# Autodesk Inventor assembly: Stadio3
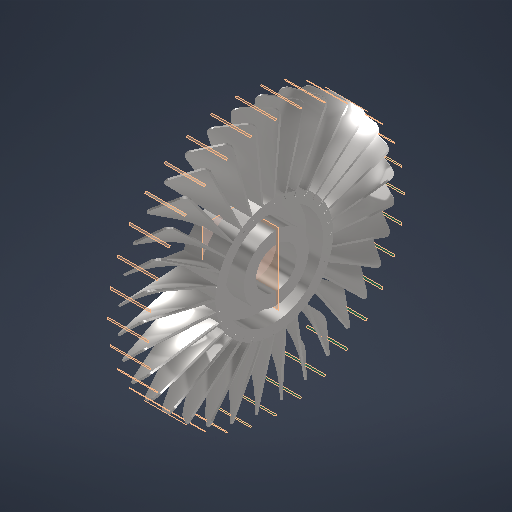
[picture p0: Inventor's stored thumbnail of the model, 512x512]
Saved by Autodesk Inventor 2026.2 (Build 302298010, 298A)
## iProperties
Created: 2026-04-23
Part Number: Stadio3
Document SubType Name: Assembly
Designer: Yan
Author: Yan
## Documents named in this file (3)
- C:\Users\Yan\Desktop\Turbina\Stadio3.iam
- C:\Users\Yan\Desktop\Turbina\DiscoPaleSatdio3-DimensioniAprossimate.ipt
- C:\Users\Yan\Desktop\Turbina\PalaStadio3.ipt
## Components (33 placed, 2 different names)
1. DiscoPaleSatdio3-DimensioniAprossimate:1 — Mate:1, Mate:3, Mate:4, Mate:5, Mate:6, Mate:7, Mate:8, Mate:9, Mate:10, Mate:11, Mate:12, Mate:13, Mate:14, Mate:15, Mate:16, Mate:17, Mate:18, Mate:19, Mate:20, Mate:21, Mate:22, Mate:23, Mate:24, Mate:25, Mate:26, Mate:27, Mate:28, Mate:29, Mate:30, Mate:31, Mate:32, Mate:33, Mate:34, Mate:35, Mate:36, Mate:37, Mate:40, Mate:41, Mate:42, Mate:43, Mate:44, Mate:45, Mate:46, Mate:47, Mate:48, Mate:49, Mate:50, Mate:51, Mate:52, Mate:53, Mate:54, Mate:55, Mate:56, Mate:57, Mate:58, Mate:59, Mate:60, Mate:61, Mate:62, Mate:63, Mate:64, Mate:65, Mate:66, Flush:1
2. PalaStadio3:1 — Mate:1, Mate:16, Flush:21
3. PalaStadio3:2 — Mate:30, Mate:31, Flush:20
4. PalaStadio3:3 — Mate:3, Mate:17, Flush:19
5. PalaStadio3:4 — Mate:4, Mate:18, Flush:18
6. PalaStadio3:5 — Mate:5, Mate:19, Flush:17
7. PalaStadio3:6 — Mate:6, Mate:20, Flush:16
8. PalaStadio3:7 — Mate:7, Mate:21, Flush:15
9. PalaStadio3:8 — Mate:8, Mate:22, Flush:14
10. PalaStadio3:9 — Mate:9, Mate:23, Flush:13
11. PalaStadio3:10 — Mate:10, Mate:24, Flush:12
12. PalaStadio3:11 — Mate:11, Mate:25, Flush:11
13. PalaStadio3:12 — Mate:58, Mate:59, Flush:32
14. PalaStadio3:13 — Mate:60, Mate:66, Flush:1, Flush:2, Flush:3, Flush:4, Flush:5, Flush:6, Flush:7, Flush:8, Flush:9, Flush:10, Flush:11, Flush:12, Flush:13, Flush:14, Flush:15, Flush:16, Flush:17, Flush:18, Flush:19, Flush:20, Flush:21, Flush:22, Flush:23, Flush:24, Flush:25, Flush:26, Flush:27, Flush:28, Flush:29, Flush:30, Flush:31, Flush:32
15. PalaStadio3:14 — Mate:37, Mate:61, Flush:2
16. PalaStadio3:15 — Mate:35, Mate:63, Flush:4
17. PalaStadio3:16 — Mate:36, Mate:64, Flush:3
18. PalaStadio3:17 — Mate:34, Mate:62, Flush:5
19. PalaStadio3:18 — Mate:32, Mate:33, Flush:6
20. PalaStadio3:19 — Mate:15, Mate:29, Flush:7
21. PalaStadio3:20 — Mate:14, Mate:28, Flush:8
22. PalaStadio3:21 — Mate:13, Mate:27, Flush:9
23. PalaStadio3:22 — Mate:12, Mate:26, Flush:10
24. PalaStadio3:24 — Mate:49, Mate:65, Flush:22
25. PalaStadio3:25 — Mate:48, Mate:50, Flush:23
26. PalaStadio3:26 — Mate:47, Mate:51, Flush:24
27. PalaStadio3:27 — Mate:46, Mate:52, Flush:25
28. PalaStadio3:28 — Mate:45, Mate:53, Flush:26
29. PalaStadio3:29 — Mate:44, Mate:54, Flush:27
30. PalaStadio3:30 — Mate:43, Mate:55, Flush:28
31. PalaStadio3:31 — Mate:42, Mate:56, Flush:29
32. PalaStadio3:32 — Mate:41, Flush:30
33. PalaStadio3:33 — Mate:40, Mate:57, Flush:31
## Relationships (95: Mate 63, Flush 32)
- Mate:1: DiscoPaleSatdio3-DimensioniAprossimate:1 ↔ PalaStadio3:1
- Mate:3: DiscoPaleSatdio3-DimensioniAprossimate:1 ↔ PalaStadio3:3
- Mate:4: DiscoPaleSatdio3-DimensioniAprossimate:1 ↔ PalaStadio3:4
- Mate:5: DiscoPaleSatdio3-DimensioniAprossimate:1 ↔ PalaStadio3:5
- Mate:6: DiscoPaleSatdio3-DimensioniAprossimate:1 ↔ PalaStadio3:6
- Mate:7: DiscoPaleSatdio3-DimensioniAprossimate:1 ↔ PalaStadio3:7
- Mate:8: DiscoPaleSatdio3-DimensioniAprossimate:1 ↔ PalaStadio3:8
- Mate:9: DiscoPaleSatdio3-DimensioniAprossimate:1 ↔ PalaStadio3:9
- Mate:10: DiscoPaleSatdio3-DimensioniAprossimate:1 ↔ PalaStadio3:10
- Mate:11: DiscoPaleSatdio3-DimensioniAprossimate:1 ↔ PalaStadio3:11
- Mate:12: DiscoPaleSatdio3-DimensioniAprossimate:1 ↔ PalaStadio3:22
- Mate:13: DiscoPaleSatdio3-DimensioniAprossimate:1 ↔ PalaStadio3:21
- Mate:14: DiscoPaleSatdio3-DimensioniAprossimate:1 ↔ PalaStadio3:20
- Mate:15: DiscoPaleSatdio3-DimensioniAprossimate:1 ↔ PalaStadio3:19
- Mate:16: DiscoPaleSatdio3-DimensioniAprossimate:1 ↔ PalaStadio3:1
- Mate:17: DiscoPaleSatdio3-DimensioniAprossimate:1 ↔ PalaStadio3:3
- Mate:18: DiscoPaleSatdio3-DimensioniAprossimate:1 ↔ PalaStadio3:4
- Mate:19: DiscoPaleSatdio3-DimensioniAprossimate:1 ↔ PalaStadio3:5
- Mate:20: DiscoPaleSatdio3-DimensioniAprossimate:1 ↔ PalaStadio3:6
- Mate:21: DiscoPaleSatdio3-DimensioniAprossimate:1 ↔ PalaStadio3:7
- Mate:22: DiscoPaleSatdio3-DimensioniAprossimate:1 ↔ PalaStadio3:8
- Mate:23: DiscoPaleSatdio3-DimensioniAprossimate:1 ↔ PalaStadio3:9
- Mate:24: DiscoPaleSatdio3-DimensioniAprossimate:1 ↔ PalaStadio3:10
- Mate:25: DiscoPaleSatdio3-DimensioniAprossimate:1 ↔ PalaStadio3:11
- Mate:26: DiscoPaleSatdio3-DimensioniAprossimate:1 ↔ PalaStadio3:22
- Mate:27: DiscoPaleSatdio3-DimensioniAprossimate:1 ↔ PalaStadio3:21
- Mate:28: DiscoPaleSatdio3-DimensioniAprossimate:1 ↔ PalaStadio3:20
- Mate:29: DiscoPaleSatdio3-DimensioniAprossimate:1 ↔ PalaStadio3:19
- Mate:30: DiscoPaleSatdio3-DimensioniAprossimate:1 ↔ PalaStadio3:2
- Mate:31: DiscoPaleSatdio3-DimensioniAprossimate:1 ↔ PalaStadio3:2
- Mate:32: DiscoPaleSatdio3-DimensioniAprossimate:1 ↔ PalaStadio3:18
- Mate:33: DiscoPaleSatdio3-DimensioniAprossimate:1 ↔ PalaStadio3:18
- Mate:34: DiscoPaleSatdio3-DimensioniAprossimate:1 ↔ PalaStadio3:17
- Mate:35: DiscoPaleSatdio3-DimensioniAprossimate:1 ↔ PalaStadio3:15
- Mate:36: DiscoPaleSatdio3-DimensioniAprossimate:1 ↔ PalaStadio3:16
- Mate:37: DiscoPaleSatdio3-DimensioniAprossimate:1 ↔ PalaStadio3:14
- Mate:40: DiscoPaleSatdio3-DimensioniAprossimate:1 ↔ PalaStadio3:33
- Mate:41: DiscoPaleSatdio3-DimensioniAprossimate:1 ↔ PalaStadio3:32
- Mate:42: DiscoPaleSatdio3-DimensioniAprossimate:1 ↔ PalaStadio3:31
- Mate:43: DiscoPaleSatdio3-DimensioniAprossimate:1 ↔ PalaStadio3:30
- Mate:44: DiscoPaleSatdio3-DimensioniAprossimate:1 ↔ PalaStadio3:29
- Mate:45: DiscoPaleSatdio3-DimensioniAprossimate:1 ↔ PalaStadio3:28
- Mate:46: DiscoPaleSatdio3-DimensioniAprossimate:1 ↔ PalaStadio3:27
- Mate:47: DiscoPaleSatdio3-DimensioniAprossimate:1 ↔ PalaStadio3:26
- Mate:48: DiscoPaleSatdio3-DimensioniAprossimate:1 ↔ PalaStadio3:25
- Mate:49: DiscoPaleSatdio3-DimensioniAprossimate:1 ↔ PalaStadio3:24
- Mate:50: DiscoPaleSatdio3-DimensioniAprossimate:1 ↔ PalaStadio3:25
- Mate:51: DiscoPaleSatdio3-DimensioniAprossimate:1 ↔ PalaStadio3:26
- Mate:52: DiscoPaleSatdio3-DimensioniAprossimate:1 ↔ PalaStadio3:27
- Mate:53: DiscoPaleSatdio3-DimensioniAprossimate:1 ↔ PalaStadio3:28
- Mate:54: DiscoPaleSatdio3-DimensioniAprossimate:1 ↔ PalaStadio3:29
- Mate:55: DiscoPaleSatdio3-DimensioniAprossimate:1 ↔ PalaStadio3:30
- Mate:56: DiscoPaleSatdio3-DimensioniAprossimate:1 ↔ PalaStadio3:31
- Mate:57: DiscoPaleSatdio3-DimensioniAprossimate:1 ↔ PalaStadio3:33
- Mate:58: DiscoPaleSatdio3-DimensioniAprossimate:1 ↔ PalaStadio3:12
- Mate:59: DiscoPaleSatdio3-DimensioniAprossimate:1 ↔ PalaStadio3:12
- Mate:60: DiscoPaleSatdio3-DimensioniAprossimate:1 ↔ PalaStadio3:13
- Mate:61: DiscoPaleSatdio3-DimensioniAprossimate:1 ↔ PalaStadio3:14
- Mate:62: DiscoPaleSatdio3-DimensioniAprossimate:1 ↔ PalaStadio3:17
- Mate:63: DiscoPaleSatdio3-DimensioniAprossimate:1 ↔ PalaStadio3:15
- Mate:64: DiscoPaleSatdio3-DimensioniAprossimate:1 ↔ PalaStadio3:16
- Mate:65: DiscoPaleSatdio3-DimensioniAprossimate:1 ↔ PalaStadio3:24
- Mate:66: DiscoPaleSatdio3-DimensioniAprossimate:1 ↔ PalaStadio3:13
- Flush:1: DiscoPaleSatdio3-DimensioniAprossimate:1 ↔ PalaStadio3:13
- Flush:2: PalaStadio3:13 ↔ PalaStadio3:14
- Flush:3: PalaStadio3:13 ↔ PalaStadio3:16
- Flush:4: PalaStadio3:13 ↔ PalaStadio3:15
- Flush:5: PalaStadio3:13 ↔ PalaStadio3:17
- Flush:6: PalaStadio3:13 ↔ PalaStadio3:18
- Flush:7: PalaStadio3:13 ↔ PalaStadio3:19
- Flush:8: PalaStadio3:13 ↔ PalaStadio3:20
- Flush:9: PalaStadio3:13 ↔ PalaStadio3:21
- Flush:10: PalaStadio3:13 ↔ PalaStadio3:22
- Flush:11: PalaStadio3:11 ↔ PalaStadio3:13
- Flush:12: PalaStadio3:10 ↔ PalaStadio3:13
- Flush:13: PalaStadio3:9 ↔ PalaStadio3:13
- Flush:14: PalaStadio3:8 ↔ PalaStadio3:13
- Flush:15: PalaStadio3:7 ↔ PalaStadio3:13
- Flush:16: PalaStadio3:6 ↔ PalaStadio3:13
- Flush:17: PalaStadio3:5 ↔ PalaStadio3:13
- Flush:18: PalaStadio3:4 ↔ PalaStadio3:13
- Flush:19: PalaStadio3:3 ↔ PalaStadio3:13
- Flush:20: PalaStadio3:2 ↔ PalaStadio3:13
- Flush:21: PalaStadio3:1 ↔ PalaStadio3:13
- Flush:22: PalaStadio3:13 ↔ PalaStadio3:24
- Flush:23: PalaStadio3:13 ↔ PalaStadio3:25
- Flush:24: PalaStadio3:13 ↔ PalaStadio3:26
- Flush:25: PalaStadio3:13 ↔ PalaStadio3:27
- Flush:26: PalaStadio3:13 ↔ PalaStadio3:28
- Flush:27: PalaStadio3:13 ↔ PalaStadio3:29
- Flush:28: PalaStadio3:13 ↔ PalaStadio3:30
- Flush:29: PalaStadio3:13 ↔ PalaStadio3:31
- Flush:30: PalaStadio3:13 ↔ PalaStadio3:32
- Flush:31: PalaStadio3:13 ↔ PalaStadio3:33
- Flush:32: PalaStadio3:12 ↔ PalaStadio3:13
